# Autodesk Inventor assembly: ASY GnG frame 1.1
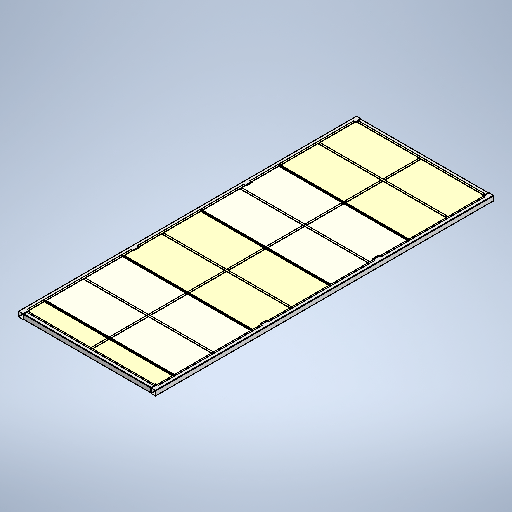
[picture p0: Inventor's stored thumbnail of the model, 512x512]
Saved by Autodesk Inventor 2025.3 (Build 293356000, 356)
## iProperties
_SolveAssemblyDoc: Frame Generator Solve Assembly
_Version: 25.0.0
Created: 2025-10-20
Part Number: ASY GnG frame 1.1
Document SubType Name: Assembly
Designer: admin
Author: admin
## Documents named in this file (8)
- C:\Users\admin\Yandex.Disk\home pc\Inventor\GnG_Gantul_hill\ASY GnG frame 1.1.iam
- C:\Users\admin\Yandex.Disk\home pc\Inventor\GnG_Gantul_hill\GnG frame 1 sketch.ipt
- C:\Users\admin\Yandex.Disk\home pc\Inventor\GnG_Gantul_hill\ASY GnG frame 1.1\Frame\Frame 1760970953553.iam
- C:\Users\admin\Yandex.Disk\home pc\Inventor\GnG_Gantul_hill\GnG frame 1.1 floor sheet.ipt
- C:\Users\admin\Yandex.Disk\home pc\Inventor\GnG_Gantul_hill\GnG frame 1.1 floor sheet 2.ipt
- C:\Users\admin\Yandex.Disk\home pc\Inventor\GnG_Gantul_hill\GnG frame 1.1 floor sheet 3.ipt
- C:\Users\admin\Yandex.Disk\home pc\Inventor\GnG_Gantul_hill\GnG frame 1.1 floor sheet 4.ipt
- C:\Users\admin\Yandex.Disk\home pc\Inventor\GnG_Gantul_hill\GnG frame 1.1 floor sheet 5.ipt
## Components (7 placed, 7 different names)
1. GnG frame 1 sketch.ipt:1
2. Frame 1760970953553.iam:1 [sub-assembly] — Flush:1, Mate:1, Mate:2
3. GnG frame 1.1 floor sheet.ipt:1 — Flush:1, Mate:1, Mate:2, Rigid:1
4. GnG frame 1.1 floor sheet 2:1 — Rigid:1, Rigid:2
5. GnG frame 1.1 floor sheet 3:1 — Rigid:2, Rigid:3
6. GnG frame 1.1 floor sheet 4:1 — Rigid:3, Rigid:4
7. GnG frame 1.1 floor sheet 5:1 — Rigid:4
## Relationships (7: WeldJoint 4, Mate 2, Flush 1)
- Flush:1: Frame 1760970953553.iam:1 ↔ GnG frame 1.1 floor sheet.ipt:1
- Mate:1 (-30 mm): Frame 1760970953553.iam:1 ↔ GnG frame 1.1 floor sheet.ipt:1
- Mate:2 (-30 mm): Frame 1760970953553.iam:1 ↔ GnG frame 1.1 floor sheet.ipt:1
- Rigid:1 [WeldJoint] (10 mm): GnG frame 1.1 floor sheet.ipt:1 ↔ GnG frame 1.1 floor sheet 2:1
- Rigid:2 [WeldJoint] (10 mm): GnG frame 1.1 floor sheet 2:1 ↔ GnG frame 1.1 floor sheet 3:1
- Rigid:3 [WeldJoint] (10 mm): GnG frame 1.1 floor sheet 3:1 ↔ GnG frame 1.1 floor sheet 4:1
- Rigid:4 [WeldJoint] (10 mm): GnG frame 1.1 floor sheet 4:1 ↔ GnG frame 1.1 floor sheet 5:1
